# Autodesk Inventor assembly: CH_00_0000_gripper
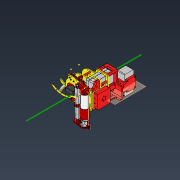
[picture p0: Inventor's stored thumbnail of the model, 180x180]
Saved by Autodesk Inventor 2022.3 (Build 263350030, 350C)
## iProperties
Created: 2022-02-10
Part Number: CH_00_0000_gripper
Document SubType Name: Assembly
Designer: Tomasz Krakowski
Author: Tomasz Krakowski
## Documents named in this file (57)
- C:\Repozytoria\sd-roboczy\01_praca\04_model\02_wykonawczy\CH_00_0000_gripper.iam
- C:\Repozytoria\sd-roboczy\01_praca\04_model\02_wykonawczy\CH_01_0001_base.ipt
- C:\Repozytoria\sd-roboczy\01_praca\04_model\02_wykonawczy\CH_01_0002_arm.ipt
- C:\Repozytoria\sd-roboczy\01_praca\04_model\02_wykonawczy\CH_01_0004_servo.ipt
- C:\Repozytoria\sd-roboczy\01_praca\04_model\02_wykonawczy\CH_01_0008_servo_horn.ipt
- C:\Repozytoria\sd-roboczy\01_praca\04_model\02_wykonawczy\CH_01_0006_syringe.ipt
- C:\Repozytoria\sd-roboczy\01_praca\04_model\02_wykonawczy\CH_01_0009_servo_shaft.ipt
- C:\Repozytoria\sd-roboczy\01_praca\04_model\02_wykonawczy\CH_01_0007_piston.ipt
- C:\Repozytoria\sd-roboczy\01_praca\04_model\02_wykonawczy\CH_01_0000_stem.ipt
- C:\Repozytoria\sd-roboczy\01_praca\04_model\02_wykonawczy\CH_01_0015_SKF_608_2RS1.ipt
- C:\Repozytoria\sd-roboczy\01_praca\04_model\02_wykonawczy\CH_01_0010_syringe_pump_servo.ipt
- C:\Repozytoria\sd-roboczy\01_praca\04_model\02_wykonawczy\CH_01_0012_bearing_plate.ipt
- C:\Repozytoria\sd-roboczy\01_praca\04_model\02_wykonawczy\CH_01_0014_syringe_mount_2.ipt
- C:\Repozytoria\sd-roboczy\01_praca\04_model\02_wykonawczy\CH_01_0016_syringe_mount_3.ipt
- C:\Repozytoria\sd-roboczy\01_praca\04_model\02_wykonawczy\CH_01_0017_distance.ipt
- C:\Repozytoria\sd-roboczy\01_praca\04_model\02_wykonawczy\CH_01_0018_arm.ipt
- C:\Repozytoria\sd-roboczy\01_praca\04_model\02_wykonawczy\CH_01_0019_bearing_plate_2.ipt
- C:\Repozytoria\sd-roboczy\01_praca\04_model\02_wykonawczy\CH_01_0020_servo_shaft_1.ipt
- C:\Repozytoria\sd-roboczy\01_praca\04_model\02_wykonawczy\CH_01_0021_distans_40mm.ipt
- C:\Repozytoria\sd-roboczy\01_praca\04_model\02_wykonawczy\CH_01_0025_end_switch.ipt
- C:\Repozytoria\sd-roboczy\01_praca\04_model\02_wykonawczy\CH_01_0025_end_switch_mount.ipt
- C:\Repozytoria\sd-roboczy\01_praca\04_model\02_wykonawczy\CH_01_0027_linear_actuator.ipt
- C:\Repozytoria\sd-roboczy\01_praca\04_model\02_wykonawczy\CH_01_0028_end_switch_mount_2.ipt
- C:\Repozytoria\sd-roboczy\01_praca\04_model\02_wykonawczy\CH_01_0029_syringe_pump_1.ipt
- C:\Repozytoria\sd-roboczy\01_praca\04_model\02_wykonawczy\CH_01_0022_bearing_mount.ipt
- C:\Repozytoria\sd-roboczy\01_praca\04_model\02_wykonawczy\CH_01_0031_bearing_mount_02.ipt
- C:\Repozytoria\sd-roboczy\01_praca\04_model\Content Center Files\en-US\DIN 912\DIN 912 - M3 x 0,5 x 8 x 6,75.ipt
- C:\Repozytoria\sd-roboczy\01_praca\04_model\Content Center Files\en-US\DIN 912\DIN 912 - M3 x 0,5 x 6 x 4,75.ipt
- C:\Repozytoria\sd-roboczy\01_praca\04_model\Content Center Files\en-US\DIN 912\DIN 912 - M3 x 0,5 x 16 x 14,75.ipt
- C:\Repozytoria\sd-roboczy\01_praca\04_model\Content Center Files\en-US\DIN 912\DIN 912 - M3 x 0,5 x 12 x 10,75.ipt
- C:\Repozytoria\sd-roboczy\01_praca\04_model\Content Center Files\en-US\PEM Concealed-head Standoffs CSS - Metric\CSS-M3-4.ipt
- C:\Repozytoria\sd-roboczy\01_praca\04_model\02_wykonawczy\CH_00_0001_needle_gripper.iam
- C:\Repozytoria\sd-roboczy\01_praca\04_model\02_wykonawczy\CH_01_0033_syringe_pump_nut_mount.ipt
- C:\Repozytoria\sd-roboczy\01_praca\04_model\02_wykonawczy\CH_01_0034_syringe_pump_nut_mount_2.ipt
- C:\Repozytoria\sd-roboczy\01_praca\04_model\Content Center Files\en-US\DIN 912\DIN 912 - M3 x 0.5 x 10 x 8.75.ipt
- C:\Repozytoria\sd-roboczy\01_praca\04_model\Content Center Files\en-US\DIN 912\DIN 912 - M3 x 0.5 x 6 x 4.75.ipt
- C:\Repozytoria\sd-roboczy\01_praca\04_model\02_wykonawczy\CH_01_0035_servo_mount.ipt
- C:\Repozytoria\sd-roboczy\01_praca\04_model\Content Center Files\en-US\DIN 912\DIN 912 - M4 x 0.7 x 8 x 6.25.ipt
- C:\Repozytoria\sd-roboczy\01_praca\04_model\Content Center Files\en-US\PEM Concealed-head Standoffs CSS - Metric\CSS-M4-4.ipt
- C:\Repozytoria\sd-roboczy\01_praca\04_model\Content Center Files\en-US\CNS 4433\CNS 4433 - M 2.ipt
- C:\Repozytoria\sd-roboczy\01_praca\04_model\Content Center Files\en-US\DIN 912\DIN 912 - M2 x 0.4 x 10 x 9.ipt
- C:\Repozytoria\sd-roboczy\01_praca\04_model\Content Center Files\en-US\DIN 912\DIN 912 - M4 x 0.7 x 40 x 20.ipt
- C:\Repozytoria\sd-roboczy\01_praca\04_model\02_wykonawczy\CH_00_0004_Z128.iam
- C:\Repozytoria\sd-roboczy\01_praca\04_model\02_wykonawczy\CH_01_0039_kradex_mount_1.ipt
- C:\Repozytoria\sd-roboczy\01_praca\04_model\02_wykonawczy\CH_01_0040_kradex_mount_2.ipt
- C:\Repozytoria\sd-roboczy\01_praca\04_model\02_wykonawczy\CH_01_0042_pcb_layout.ipt
- C:\Repozytoria\sd-roboczy\01_praca\04_model\02_wykonawczy\CH_01_0044_motor_end.ipt
- C:\Repozytoria\sd-roboczy\01_praca\04_model\02_wykonawczy\CH_01_0045_endefector_mount.ipt
- C:\Repozytoria\sd-roboczy\01_praca\04_model\02_wykonawczy\CH_01_0046_arm.ipt
- C:\Repozytoria\sd-roboczy\01_praca\04_model\02_wykonawczy\CH_01_0047_camera_mount.ipt
- C:\Repozytoria\sd-roboczy\01_praca\04_model\02_wykonawczy\CH_01_0043_camera_PH.ipt
- C:\Repozytoria\sd-roboczy\01_praca\04_model\02_wykonawczy\CH_01_0049_distans_40mm.ipt
- C:\Repozytoria\sd-roboczy\01_praca\04_model\02_wykonawczy\CH_01_0050_distans_40mm.ipt
- C:\Repozytoria\sd-roboczy\01_praca\04_model\02_wykonawczy\CH_01_0011_syringe_pump_needle mount_lower.ipt
- C:\Repozytoria\sd-roboczy\01_praca\04_model\02_wykonawczy\CH_01_0052_bracket_mount.ipt
- C:\Repozytoria\sd-roboczy\01_praca\04_model\02_wykonawczy\CH_01_0053_camera_mount.ipt
- C:\Repozytoria\sd-roboczy\01_praca\04_model\02_wykonawczy\CH_01_0054_camer_mount_part_b.ipt
## Components (121 placed, 55 different names)
1. CH_01_0001_base:1 — Mate:25, Mate:26, Mate:27, Zestawiający:43, pompa:51, Mate:53, Mate:54, Mate:58, Zestawiający:66, Zestawiający:73, Mate:94, Mate:100, Mate:102, Mate:103, Mate:106, Mate:115, Mate:164, Mate:165, Mate:166, Mate:169, Mate:170, Mate:171, Mate:172, Mate:179, Mate:180, Mate:181, Mate:182, Mate:193, Mate:194, Mate:196, Mate:225, Mate:226, Mate:289, Mate:290, Mate:292, Mate:295
2. CH_01_0002_arm:1 — Mate:17, Mate:18, Mate:19, Mate:30, Mate:32
3. CH_01_0006_syringe:1 — Mate:22, Mate:23, Zestawiający:49, Zestawiający:50, Mate:134, Mate:136
4. CH_01_0007_piston:1 — Mate:22, Mate:23, Mate:126, Mate:127, Mate:137, Flush:18
5. CH_01_0000_stem:1 — Mate:25
6. CH_01_0004_servo:1 — Mate:26, Mate:27, Mate:28, Mate:29, Mate:58
7. CH_01_0008_servo_horn:2 — Mate:28, Mate:29, Mate:30, Mate:31, Mate:32
8. SKF 2RS1-  with two seals SKF 2RS1608-2RS1:1 — Zestawiający:34, Mate:57, Mate:131
9. CH_01_0012_bearing_plate:1 — Zestawiający:43, Zestawiający:63, Zestawiający:64, Zestawiający:65, Zestawiający:66, Zestawiający:79, Zestawiający:80, Mate:101, Mate:110, Mate:112, Mate:113, Mate:114, Mate:132, Mate:133, Mate:233, Mate:234, Mate:235, Mate:236, Mate:237, Mate:238, Mate:246, Mate:251, Mate:252, Mate:253, Mate:254, Mate:259, Flush:48, Flush:49, Mate:281, Mate:282, Mate:283, Mate:284, Mate:285, Mate:286, Mate:287, Mate:288
10. CH_01_0014_syringe_mount_2:1 — Zestawiający:49, Zestawiający:50, pompa:51, Zestawiający:73, Mate:124, Mate:125, Mate:155, Flush:24, Mate:156, Flush:25, Mate:157
11. CH_01_0016_syringe_mount_3:1 — Mate:53, Mate:54, Mate:134, Mate:135, Flush:18, Mate:149, Mate:150, Mate:154, Flush:23, Mate:158, Mate:159
12. CH_01_0017_distance:1 — Mate:56, Mate:57, Zestawiający:62
13. CH_01_0018_arm:1 — Zestawiający:59, Zestawiający:60, Zestawiający:61
14. SKF 2RS1-  with two seals SKF 2RS1608-2RS1:2 — Zestawiający:62, Zestawiający:63, Równoległy:4, Mate:128, Mate:129
15. CH_01_0019_bearing_plate_2:1 — Zestawiający:64, Zestawiający:65, Równoległy:4, Zestawiający:82, Zestawiający:83, Mate:119, Mate:122, Flush:17, Mate:123, Mate:130, Mate:228, Mate:229, Mate:230, Mate:231, Mate:232, Mate:250, Mate:261, Mate:264, Mate:265, Mate:266, Mate:303, Flush:53, Flush:54
16. CH_01_0020_servo_shaft_1:1 — Zestawiający:67, Zestawiający:68, Mate:142
17. CH_01_0021_distans_40mm:3 — Zestawiający:79, Zestawiający:82, Mate:111, Flush:13
18. CH_01_0021_distans_40mm:4 — Zestawiający:80, Zestawiający:83, Mate:111, Flush:14
19. CH_01_0025_end_switch:1 — Mate:95, Mate:96, Mate:97, Mate:215, Mate:216, Mate:217
20. CH_01_0025_end_switch_mount:1 — Mate:94, Mate:95, Mate:96, Mate:97, Mate:102, Mate:103, Mate:177, Flush:28, Mate:178, Flush:29, Mate:202, Flush:35, Mate:203, Flush:36
21. CH_01_0027_linear_actuator:1 — Mate:124, Mate:125, Flush:25, Mate:296
22. CH_01_0021_distans_40mm:6 — Mate:100, Mate:101
23. CH_01_0028_end_switch_mount_2:1 — Mate:106, Mate:107, Mate:108, Mate:109, Mate:173, Flush:26, Mate:174, Flush:27, Mate:204, Mate:205, Flush:37, Flush:38
24. CH_01_0025_end_switch:2 — Mate:107, Mate:108, Mate:109, Mate:218, Mate:219, Mate:220
25. CH_01_0021_distans_40mm:7 — Mate:110, Flush:13, Mate:112, Mate:115
26. CH_01_0021_distans_40mm:8 — Mate:113, Flush:14, Mate:114
27. CH_01_0021_distans_40mm:9 — Mate:119, Mate:122, Mate:227
28. CH_01_0010_syringe_pump_servo:1 — Flush:17, Mate:123, Mate:246, Mate:267, Mate:268, Mate:269, Mate:298, Mate:299, Mate:300, Mate:301, Mate:302
29. CH_01_0029_syringe_pump_1:1 — Mate:126, Mate:127, Mate:137, Mate:143, Mate:145, Flush:20, Mate:297
30. CH_01_0022_bearing_mount:1 — Mate:128, Mate:129, Mate:130, Mate:221, Flush:41, Mate:222, Flush:42
31. CH_01_0031_bearing_mount_02:1 — Mate:131, Mate:132, Mate:133, Mate:223, Mate:224, Flush:43, Flush:44
32. DIN 912 - replaced by DIN EN ISO 4762 M3 x 8:1 — Mate:135, Mate:136
33. DIN 912 - replaced by DIN EN ISO 4762 M3 x 6:1 — Mate:143, Mate:152
34. DIN 912 - replaced by DIN EN ISO 4762 M3 x 6:2 — Mate:145, Mate:153
35. DIN 912 - replaced by DIN EN ISO 4762 M3 x 16:1 — Mate:296, Mate:297
36. DIN 912 - replaced by DIN EN ISO 4762 M3 x 12:1 — Mate:149, Mate:150, Mate:168
37. PEM Concealed-head Standoffs CSS - Metric CSS-M3-4:1 — Flush:20
38. PEM Concealed-head Standoffs CSS - Metric CSS-M3-4:3 — Mate:152
39. PEM Concealed-head Standoffs CSS - Metric CSS-M3-4:4 — Mate:153
40. PEM Concealed-head Standoffs CSS - Metric CSS-M3-4:5 — Mate:154, Flush:23
41. PEM Concealed-head Standoffs CSS - Metric CSS-M3-4:6 — Mate:155, Flush:24
42. DIN 912 - replaced by DIN EN ISO 4762 M3 x 16:3 — Mate:156, Mate:157
43. DIN 912 - replaced by DIN EN ISO 4762 M3 x 12:2 — Mate:158, Mate:159, Mate:167
44. DIN 912 - replaced by DIN EN ISO 4762 M3 x 10:2 — Mate:176
45. DIN 912 - replaced by DIN EN ISO 4762 M3 x 10:1 — Mate:175
46. CH_00_0001_needle_gripper:1 [sub-assembly] — Mate:164, Mate:165, Mate:166, Mate:185, Mate:186, Mate:187, Mate:188
47. CH_01_0033_syringe_pump_nut_mount:1 — Mate:167, Mate:168, Mate:169
48. CH_01_0034_syringe_pump_nut_mount_2:1 — Mate:170, Mate:171, Mate:172, Mate:183, Flush:30, Mate:184, Flush:31
49. PEM Concealed-head Standoffs CSS - Metric CSS-M3-4:7 — Mate:174, Flush:27, Mate:175
50. PEM Concealed-head Standoffs CSS - Metric CSS-M3-4:8 — Mate:173, Flush:26, Mate:176
51. PEM Concealed-head Standoffs CSS - Metric CSS-M3-4:9 — Mate:178, Flush:29
52. PEM Concealed-head Standoffs CSS - Metric CSS-M3-4:10 — Mate:177, Flush:28
53. DIN 912 - replaced by DIN EN ISO 4762 M3 x 6:3 — Mate:179, Mate:181
54. DIN 912 - replaced by DIN EN ISO 4762 M3 x 6:4 — Mate:180, Mate:182
55. PEM Concealed-head Standoffs CSS - Metric CSS-M3-4:11 — Mate:183, Flush:30
56. PEM Concealed-head Standoffs CSS - Metric CSS-M3-4:12 — Mate:184, Flush:31
57. DIN 912 - replaced by DIN EN ISO 4762 M3 x 10:3 — Mate:185, Mate:186, Mate:293
58. DIN 912 - replaced by DIN EN ISO 4762 M3 x 10:4 — Mate:187, Mate:188, Mate:294
59. CH_01_0035_servo_mount:1 — Mate:193, Mate:194, Mate:195, Mate:196, Flush:34
60. CNS 4433 M 2:1 — Mate:202, Flush:35
61. CNS 4433 M 2:3 — Mate:203, Flush:36
62. CNS 4433 M 2:4 — Mate:204, Flush:37
63. CNS 4433 M 2:5 — Mate:205, Flush:38
64. DIN 912 - replaced by DIN EN ISO 4762 M2 x 10:1 — Mate:215, Flush:39, Mate:217
65. DIN 912 - replaced by DIN EN ISO 4762 M2 x 10:2 — Mate:216, Flush:39
66. DIN 912 - replaced by DIN EN ISO 4762 M2 x 10:3 — Mate:218, Flush:40, Mate:220
67. DIN 912 - replaced by DIN EN ISO 4762 M2 x 10:4 — Mate:219, Flush:40
68. PEM Concealed-head Standoffs CSS - Metric CSS-M3-4:15 — Mate:221, Flush:41
69. PEM Concealed-head Standoffs CSS - Metric CSS-M3-4:16 — Mate:222, Flush:42
70. PEM Concealed-head Standoffs CSS - Metric CSS-M3-4:17 — Mate:223, Flush:43
71. PEM Concealed-head Standoffs CSS - Metric CSS-M3-4:18 — Mate:224, Flush:44
72. DIN 912 - replaced by DIN EN ISO 4762 M3 x 6:9 — Mate:225, Mate:226
73. DIN 912 - replaced by DIN EN ISO 4762 M3 x 6:14 — Mate:229, Mate:230
74. DIN 912 - replaced by DIN EN ISO 4762 M3 x 6:15 — Mate:231, Mate:232
75. DIN 912 - replaced by DIN EN ISO 4762 M3 x 6:16 — Mate:233, Flush:45
76. DIN 912 - replaced by DIN EN ISO 4762 M3 x 6:17 — Mate:234, Flush:45, Mate:235
77. CH_00_0001_needle_gripper:2 [sub-assembly] — Mate:236, Mate:237, Mate:238
78. CH_00_0004_Z128:1 [sub-assembly] — Mate:261, Mate:262, Flush:50, Mate:263, Mate:266, Flush:51
79. CH_01_0039_kradex_mount_1:1 — Mate:250, Mate:255, Mate:256, Mate:257, Flush:51
80. DIN 912 - replaced by DIN EN ISO 4762 M3 x 10:5 — Mate:251, Mate:253
81. DIN 912 - replaced by DIN EN ISO 4762 M3 x 10:6 — Mate:252, Mate:254
82. DIN 912 - replaced by DIN EN ISO 4762 M3 x 10:7 — Mate:255, Flush:47, Mate:264
83. DIN 912 - replaced by DIN EN ISO 4762 M3 x 10:8 — Mate:256, Flush:47, Mate:257, Mate:265
84. CH_01_0040_kradex_mount_2:1 — Mate:259, Flush:48, Flush:49
85. CH_01_0042_pcb_layout:1 — Mate:262, Flush:50, Mate:263
86. CH_01_0044_motor_end:1 — Mate:270, Mate:271, Mate:272, Mate:273, Mate:274, Mate:277, Mate:278
87. CH_01_0045_endefector_mount:1 — Mate:267, Mate:268, Mate:269, Mate:270, Mate:271, Mate:272
88. CH_01_0046_arm:1 — Mate:273, Mate:274, Mate:275, Mate:276, Mate:277
89. CH_01_0047_camera_mount:1 — Mate:275, Mate:276, Mate:278
90. CH_01_0043_camera_PH:1 — Mate:304, Mate:305, Mate:306
91. CH_01_0049_distans_40mm:1 — Mate:281, Mate:287
92. CH_01_0049_distans_40mm:2 — Mate:282, Mate:288
93. CH_01_0049_distans_40mm:3 — Mate:283, Mate:284
94. CH_01_0049_distans_40mm:4 — Mate:285, Mate:286
95. CH_01_0050_distans_40mm:1 — Mate:290, Mate:291, Mate:292
96. CH_01_0050_distans_40mm:2 — Mate:289, Mate:291
97. CH_01_0011_syringe_pump_needle mount_lower:1 — Mate:293, Mate:294, Mate:295
98. CH_01_0052_bracket_mount:1 — Mate:298, Mate:301
99. CH_01_0052_bracket_mount:2 — Mate:299, Mate:300, Mate:302
100. CH_01_0053_camera_mount:1 — Mate:303, Flush:53, Flush:54, Mate:307, Mate:308
101. CH_01_0054_camer_mount_part_b:1 — Mate:304, Mate:305, Mate:306, Mate:307, Mate:308
102. DIN 912 - replaced by DIN EN ISO 4762 M3 x 6:5 — Mate:191, Mate:192
103. CH_01_0009_servo_shaft:1 — Mate:17, Mate:18, Mate:19, Mate:31, Zestawiający:34, Mate:56, Zestawiający:59, Zestawiający:60, Zestawiający:61, Zestawiający:67, Zestawiający:68, Mate:142, Mate:191, Mate:192
104. DIN 912 - replaced by DIN EN ISO 4762 M3 x 6:6
105. CH_01_0009_servo_shaft:2
106. DIN 912 - replaced by DIN EN ISO 4762 M3 x 6:7
107. CH_01_0009_servo_shaft:3
108. DIN 912 - replaced by DIN EN ISO 4762 M3 x 6:8
109. CH_01_0009_servo_shaft:4
110. PEM Concealed-head Standoffs CSS - Metric CSS-M4-4:1 — Mate:195, Flush:34
111. PEM Concealed-head Standoffs CSS - Metric CSS-M4-4:2
112. PEM Concealed-head Standoffs CSS - Metric CSS-M4-4:3
113. PEM Concealed-head Standoffs CSS - Metric CSS-M4-4:4
114. DIN 912 - replaced by DIN EN ISO 4762 M4 x 8:1
115. DIN 912 - replaced by DIN EN ISO 4762 M4 x 8:2
116. DIN 912 - replaced by DIN EN ISO 4762 M4 x 8:3
117. DIN 912 - replaced by DIN EN ISO 4762 M4 x 8:4
118. DIN 912 - replaced by DIN EN ISO 4762 M4 x 40:1 — Mate:227, Mate:228
119. DIN 912 - replaced by DIN EN ISO 4762 M4 x 40:2
120. DIN 912 - replaced by DIN EN ISO 4762 M4 x 40:3
121. DIN 912 - replaced by DIN EN ISO 4762 M4 x 40:4
## Component patterns: (4 elements, first: DIN 912 - replaced by DIN EN ISO 4762 M3 x 6:5 + CH_01_0009_servo_shaft:1), (4 elements, first: PEM Concealed-head Standoffs CSS - Metric CSS-M4-4:1), (4 elements, first: DIN 912 - replaced by DIN EN ISO 4762 M4 x 8:1), (4 elements, first: DIN 912 - replaced by DIN EN ISO 4762 M4 x 40:1)
## Relationships (240: Mate 206, Flush 34)
- Mate:17: CH_01_0002_arm:1 ↔ CH_01_0009_servo_shaft:1
- Mate:18: CH_01_0002_arm:1 ↔ CH_01_0009_servo_shaft:1
- Mate:19: CH_01_0002_arm:1 ↔ CH_01_0009_servo_shaft:1
- Mate:22: CH_01_0006_syringe:1 ↔ CH_01_0007_piston:1
- Mate:23: CH_01_0006_syringe:1 ↔ CH_01_0007_piston:1
- Mate:25: CH_01_0001_base:1 ↔ CH_01_0000_stem:1
- Mate:26: CH_01_0001_base:1 ↔ CH_01_0004_servo:1
- Mate:27: CH_01_0001_base:1 ↔ CH_01_0004_servo:1
- Mate:28: CH_01_0004_servo:1 ↔ CH_01_0008_servo_horn:2
- Mate:29: CH_01_0004_servo:1 ↔ CH_01_0008_servo_horn:2
- Mate:30: CH_01_0002_arm:1 ↔ CH_01_0008_servo_horn:2
- Mate:31: CH_01_0008_servo_horn:2 ↔ CH_01_0009_servo_shaft:1
- Mate:32: CH_01_0002_arm:1 ↔ CH_01_0008_servo_horn:2
- Zestawiający:34 [Mate]: SKF 2RS1-  with two seals SKF 2RS1608-2RS1:1 ↔ CH_01_0009_servo_shaft:1
- Zestawiający:43 [Mate]: CH_01_0001_base:1 ↔ CH_01_0012_bearing_plate:1
- Zestawiający:49 [Mate]: CH_01_0006_syringe:1 ↔ CH_01_0014_syringe_mount_2:1
- Zestawiający:50 [Mate]: CH_01_0006_syringe:1 ↔ CH_01_0014_syringe_mount_2:1
- pompa:51 [Mate] (4 mm): CH_01_0001_base:1 ↔ CH_01_0014_syringe_mount_2:1
- Mate:53: CH_01_0001_base:1 ↔ CH_01_0016_syringe_mount_3:1
- Mate:54: CH_01_0001_base:1 ↔ CH_01_0016_syringe_mount_3:1
- Mate:56: CH_01_0017_distance:1 ↔ CH_01_0009_servo_shaft:1
- Mate:57: SKF 2RS1-  with two seals SKF 2RS1608-2RS1:1 ↔ CH_01_0017_distance:1
- Mate:58: CH_01_0001_base:1 ↔ CH_01_0004_servo:1
- Zestawiający:59 [Mate]: CH_01_0018_arm:1 ↔ CH_01_0009_servo_shaft:1
- Zestawiający:60 [Mate]: CH_01_0018_arm:1 ↔ CH_01_0009_servo_shaft:1
- Zestawiający:61 [Mate]: CH_01_0018_arm:1 ↔ CH_01_0009_servo_shaft:1
- Zestawiający:62 [Mate]: CH_01_0017_distance:1 ↔ SKF 2RS1-  with two seals SKF 2RS1608-2RS1:2
- Zestawiający:63 [Mate] (40 mm): CH_01_0012_bearing_plate:1 ↔ SKF 2RS1-  with two seals SKF 2RS1608-2RS1:2
- Zestawiający:64 [Mate]: CH_01_0012_bearing_plate:1 ↔ CH_01_0019_bearing_plate_2:1
- Zestawiający:65 [Mate]: CH_01_0012_bearing_plate:1 ↔ CH_01_0019_bearing_plate_2:1
- Zestawiający:66 [Mate]: CH_01_0001_base:1 ↔ CH_01_0012_bearing_plate:1
- Równoległy:4 [Flush]: SKF 2RS1-  with two seals SKF 2RS1608-2RS1:2 ↔ CH_01_0019_bearing_plate_2:1
- Zestawiający:67 [Mate]: CH_01_0020_servo_shaft_1:1 ↔ CH_01_0009_servo_shaft:1
- Zestawiający:68 [Mate]: CH_01_0020_servo_shaft_1:1 ↔ CH_01_0009_servo_shaft:1
- Zestawiający:73 [Mate]: CH_01_0001_base:1 ↔ CH_01_0014_syringe_mount_2:1
- Zestawiający:79 [Mate]: CH_01_0012_bearing_plate:1 ↔ CH_01_0021_distans_40mm:3
- Zestawiający:80 [Mate]: CH_01_0012_bearing_plate:1 ↔ CH_01_0021_distans_40mm:4
- Zestawiający:82 [Mate]: CH_01_0019_bearing_plate_2:1 ↔ CH_01_0021_distans_40mm:3
- Zestawiający:83 [Mate]: CH_01_0019_bearing_plate_2:1 ↔ CH_01_0021_distans_40mm:4
- Mate:94: CH_01_0001_base:1 ↔ CH_01_0025_end_switch_mount:1
- Mate:95: CH_01_0025_end_switch:1 ↔ CH_01_0025_end_switch_mount:1
- Mate:96: CH_01_0025_end_switch:1 ↔ CH_01_0025_end_switch_mount:1
- Mate:97: CH_01_0025_end_switch:1 ↔ CH_01_0025_end_switch_mount:1
- Mate:100: CH_01_0001_base:1 ↔ CH_01_0021_distans_40mm:6
- Mate:101: CH_01_0012_bearing_plate:1 ↔ CH_01_0021_distans_40mm:6
- Mate:102: CH_01_0001_base:1 ↔ CH_01_0025_end_switch_mount:1
- Mate:103: CH_01_0001_base:1 ↔ CH_01_0025_end_switch_mount:1
- Mate:106: CH_01_0001_base:1 ↔ CH_01_0028_end_switch_mount_2:1
- Mate:107: CH_01_0028_end_switch_mount_2:1 ↔ CH_01_0025_end_switch:2
- Mate:108: CH_01_0028_end_switch_mount_2:1 ↔ CH_01_0025_end_switch:2
- Mate:109: CH_01_0028_end_switch_mount_2:1 ↔ CH_01_0025_end_switch:2
- Mate:110: CH_01_0012_bearing_plate:1 ↔ CH_01_0021_distans_40mm:7
- Mate:111: CH_01_0021_distans_40mm:3 ↔ CH_01_0021_distans_40mm:4
- Flush:13: CH_01_0021_distans_40mm:3 ↔ CH_01_0021_distans_40mm:7
- Mate:112: CH_01_0012_bearing_plate:1 ↔ CH_01_0021_distans_40mm:7
- Mate:113: CH_01_0012_bearing_plate:1 ↔ CH_01_0021_distans_40mm:8
- Flush:14: CH_01_0021_distans_40mm:4 ↔ CH_01_0021_distans_40mm:8
- Mate:114: CH_01_0012_bearing_plate:1 ↔ CH_01_0021_distans_40mm:8
- Mate:115: CH_01_0001_base:1 ↔ CH_01_0021_distans_40mm:7
- Mate:119: CH_01_0019_bearing_plate_2:1 ↔ CH_01_0021_distans_40mm:9
- Mate:122: CH_01_0019_bearing_plate_2:1 ↔ CH_01_0021_distans_40mm:9
- Flush:17: CH_01_0019_bearing_plate_2:1 ↔ CH_01_0010_syringe_pump_servo:1
- Mate:123: CH_01_0019_bearing_plate_2:1 ↔ CH_01_0010_syringe_pump_servo:1
- Mate:124: CH_01_0014_syringe_mount_2:1 ↔ CH_01_0027_linear_actuator:1
- Mate:125: CH_01_0014_syringe_mount_2:1 ↔ CH_01_0027_linear_actuator:1
- Mate:126: CH_01_0007_piston:1 ↔ CH_01_0029_syringe_pump_1:1
- Mate:127: CH_01_0007_piston:1 ↔ CH_01_0029_syringe_pump_1:1
- Mate:128: SKF 2RS1-  with two seals SKF 2RS1608-2RS1:2 ↔ CH_01_0022_bearing_mount:1
- Mate:129: SKF 2RS1-  with two seals SKF 2RS1608-2RS1:2 ↔ CH_01_0022_bearing_mount:1
- Mate:130: CH_01_0019_bearing_plate_2:1 ↔ CH_01_0022_bearing_mount:1
- Mate:131: SKF 2RS1-  with two seals SKF 2RS1608-2RS1:1 ↔ CH_01_0031_bearing_mount_02:1
- Mate:132: CH_01_0012_bearing_plate:1 ↔ CH_01_0031_bearing_mount_02:1
- Mate:133: CH_01_0012_bearing_plate:1 ↔ CH_01_0031_bearing_mount_02:1
- Mate:134: CH_01_0006_syringe:1 ↔ CH_01_0016_syringe_mount_3:1
- Mate:135: CH_01_0016_syringe_mount_3:1 ↔ DIN 912 - replaced by DIN EN ISO 4762 M3 x 8:1
- Mate:136: CH_01_0006_syringe:1 ↔ DIN 912 - replaced by DIN EN ISO 4762 M3 x 8:1
- Mate:137: CH_01_0007_piston:1 ↔ CH_01_0029_syringe_pump_1:1
- Flush:18: CH_01_0007_piston:1 ↔ CH_01_0016_syringe_mount_3:1
- Mate:142: CH_01_0020_servo_shaft_1:1 ↔ CH_01_0009_servo_shaft:1
- Mate:143: CH_01_0029_syringe_pump_1:1 ↔ DIN 912 - replaced by DIN EN ISO 4762 M3 x 6:1
- Mate:145: CH_01_0029_syringe_pump_1:1 ↔ DIN 912 - replaced by DIN EN ISO 4762 M3 x 6:2
- Mate:149: CH_01_0016_syringe_mount_3:1 ↔ DIN 912 - replaced by DIN EN ISO 4762 M3 x 12:1
- Mate:150: CH_01_0016_syringe_mount_3:1 ↔ DIN 912 - replaced by DIN EN ISO 4762 M3 x 12:1
- Flush:20 (0.1 mm): CH_01_0029_syringe_pump_1:1 ↔ PEM Concealed-head Standoffs CSS - Metric CSS-M3-4:1
- Mate:152: DIN 912 - replaced by DIN EN ISO 4762 M3 x 6:1 ↔ PEM Concealed-head Standoffs CSS - Metric CSS-M3-4:3
- Mate:153: DIN 912 - replaced by DIN EN ISO 4762 M3 x 6:2 ↔ PEM Concealed-head Standoffs CSS - Metric CSS-M3-4:4
- Mate:154: CH_01_0016_syringe_mount_3:1 ↔ PEM Concealed-head Standoffs CSS - Metric CSS-M3-4:5
- Flush:23 (0.1 mm): CH_01_0016_syringe_mount_3:1 ↔ PEM Concealed-head Standoffs CSS - Metric CSS-M3-4:5
- Mate:155: CH_01_0014_syringe_mount_2:1 ↔ PEM Concealed-head Standoffs CSS - Metric CSS-M3-4:6
- Flush:24 (0.1 mm): CH_01_0014_syringe_mount_2:1 ↔ PEM Concealed-head Standoffs CSS - Metric CSS-M3-4:6
- Mate:156: CH_01_0014_syringe_mount_2:1 ↔ DIN 912 - replaced by DIN EN ISO 4762 M3 x 16:3
- Flush:25: CH_01_0014_syringe_mount_2:1 ↔ CH_01_0027_linear_actuator:1
- Mate:157: CH_01_0014_syringe_mount_2:1 ↔ DIN 912 - replaced by DIN EN ISO 4762 M3 x 16:3
- Mate:158: CH_01_0016_syringe_mount_3:1 ↔ DIN 912 - replaced by DIN EN ISO 4762 M3 x 12:2
- Mate:159: CH_01_0016_syringe_mount_3:1 ↔ DIN 912 - replaced by DIN EN ISO 4762 M3 x 12:2
- [Mate]: CH_01_0014_syringe_mount_2:1 ↔ DIN 912 - replaced by DIN EN ISO 4762 M3 x 10:1
- [Mate]: CH_01_0014_syringe_mount_2:1 ↔ DIN 912 - replaced by DIN EN ISO 4762 M3 x 10:2
- [Mate]: CH_01_0014_syringe_mount_2:1 ↔ DIN 912 - replaced by DIN EN ISO 4762 M3 x 10:1
- [Mate]: CH_01_0014_syringe_mount_2:1 ↔ DIN 912 - replaced by DIN EN ISO 4762 M3 x 10:2
- Mate:164: CH_01_0001_base:1 ↔ CH_00_0001_needle_gripper:1
- Mate:165: CH_01_0001_base:1 ↔ CH_00_0001_needle_gripper:1
- Mate:166: CH_01_0001_base:1 ↔ CH_00_0001_needle_gripper:1
- Mate:167: DIN 912 - replaced by DIN EN ISO 4762 M3 x 12:2 ↔ CH_01_0033_syringe_pump_nut_mount:1
- Mate:168: DIN 912 - replaced by DIN EN ISO 4762 M3 x 12:1 ↔ CH_01_0033_syringe_pump_nut_mount:1
- Mate:169: CH_01_0001_base:1 ↔ CH_01_0033_syringe_pump_nut_mount:1
- Mate:170: CH_01_0001_base:1 ↔ CH_01_0034_syringe_pump_nut_mount_2:1
- Mate:171: CH_01_0001_base:1 ↔ CH_01_0034_syringe_pump_nut_mount_2:1
- Mate:172: CH_01_0001_base:1 ↔ CH_01_0034_syringe_pump_nut_mount_2:1
- Mate:173: CH_01_0028_end_switch_mount_2:1 ↔ PEM Concealed-head Standoffs CSS - Metric CSS-M3-4:8
- Flush:26 (0.1 mm): CH_01_0028_end_switch_mount_2:1 ↔ PEM Concealed-head Standoffs CSS - Metric CSS-M3-4:8
- Mate:174: CH_01_0028_end_switch_mount_2:1 ↔ PEM Concealed-head Standoffs CSS - Metric CSS-M3-4:7
- Flush:27 (0.1 mm): CH_01_0028_end_switch_mount_2:1 ↔ PEM Concealed-head Standoffs CSS - Metric CSS-M3-4:7
- Mate:175: DIN 912 - replaced by DIN EN ISO 4762 M3 x 10:1 ↔ PEM Concealed-head Standoffs CSS - Metric CSS-M3-4:7
- Mate:176: DIN 912 - replaced by DIN EN ISO 4762 M3 x 10:2 ↔ PEM Concealed-head Standoffs CSS - Metric CSS-M3-4:8
- Mate:177: CH_01_0025_end_switch_mount:1 ↔ PEM Concealed-head Standoffs CSS - Metric CSS-M3-4:10
- Flush:28 (0.1 mm): CH_01_0025_end_switch_mount:1 ↔ PEM Concealed-head Standoffs CSS - Metric CSS-M3-4:10
- Mate:178: CH_01_0025_end_switch_mount:1 ↔ PEM Concealed-head Standoffs CSS - Metric CSS-M3-4:9
- Flush:29 (0.1 mm): CH_01_0025_end_switch_mount:1 ↔ PEM Concealed-head Standoffs CSS - Metric CSS-M3-4:9
- Mate:179: CH_01_0001_base:1 ↔ DIN 912 - replaced by DIN EN ISO 4762 M3 x 6:3
- Mate:180: CH_01_0001_base:1 ↔ DIN 912 - replaced by DIN EN ISO 4762 M3 x 6:4
- Mate:181: CH_01_0001_base:1 ↔ DIN 912 - replaced by DIN EN ISO 4762 M3 x 6:3
- Mate:182: CH_01_0001_base:1 ↔ DIN 912 - replaced by DIN EN ISO 4762 M3 x 6:4
- Mate:183: CH_01_0034_syringe_pump_nut_mount_2:1 ↔ PEM Concealed-head Standoffs CSS - Metric CSS-M3-4:11
- Flush:30 (0.1 mm): CH_01_0034_syringe_pump_nut_mount_2:1 ↔ PEM Concealed-head Standoffs CSS - Metric CSS-M3-4:11
- Mate:184: CH_01_0034_syringe_pump_nut_mount_2:1 ↔ PEM Concealed-head Standoffs CSS - Metric CSS-M3-4:12
- Flush:31 (0.1 mm): CH_01_0034_syringe_pump_nut_mount_2:1 ↔ PEM Concealed-head Standoffs CSS - Metric CSS-M3-4:12
- Mate:185: CH_00_0001_needle_gripper:1 ↔ DIN 912 - replaced by DIN EN ISO 4762 M3 x 10:3
- Mate:186: CH_00_0001_needle_gripper:1 ↔ DIN 912 - replaced by DIN EN ISO 4762 M3 x 10:3
- Mate:187: CH_00_0001_needle_gripper:1 ↔ DIN 912 - replaced by DIN EN ISO 4762 M3 x 10:4
- Mate:188: CH_00_0001_needle_gripper:1 ↔ DIN 912 - replaced by DIN EN ISO 4762 M3 x 10:4
- Mate:191: DIN 912 - replaced by DIN EN ISO 4762 M3 x 6:5 ↔ CH_01_0009_servo_shaft:1
- Mate:192: DIN 912 - replaced by DIN EN ISO 4762 M3 x 6:5 ↔ CH_01_0009_servo_shaft:1
- Mate:193: CH_01_0001_base:1 ↔ CH_01_0035_servo_mount:1
- Mate:194: CH_01_0001_base:1 ↔ CH_01_0035_servo_mount:1
- Mate:195: CH_01_0035_servo_mount:1 ↔ PEM Concealed-head Standoffs CSS - Metric CSS-M4-4:1
- Mate:196: CH_01_0001_base:1 ↔ CH_01_0035_servo_mount:1
- Flush:34 (0.1 mm): CH_01_0035_servo_mount:1 ↔ PEM Concealed-head Standoffs CSS - Metric CSS-M4-4:1
- [Mate]: CH_01_0001_base:1 ↔ DIN 912 - replaced by DIN EN ISO 4762 M4 x 8:1
- Mate:202: CH_01_0025_end_switch_mount:1 ↔ CNS 4433 M 2:1
- Flush:35 (0.1 mm): CH_01_0025_end_switch_mount:1 ↔ CNS 4433 M 2:1
- Mate:203: CH_01_0025_end_switch_mount:1 ↔ CNS 4433 M 2:3
- Flush:36 (0.1 mm): CH_01_0025_end_switch_mount:1 ↔ CNS 4433 M 2:3
- Mate:204: CH_01_0028_end_switch_mount_2:1 ↔ CNS 4433 M 2:4
- Mate:205: CH_01_0028_end_switch_mount_2:1 ↔ CNS 4433 M 2:5
- Flush:37 (0.1 mm): CH_01_0028_end_switch_mount_2:1 ↔ CNS 4433 M 2:4
- Flush:38 (0.1 mm): CH_01_0028_end_switch_mount_2:1 ↔ CNS 4433 M 2:5
- Mate:215: CH_01_0025_end_switch:1 ↔ DIN 912 - replaced by DIN EN ISO 4762 M2 x 10:1
- Mate:216: CH_01_0025_end_switch:1 ↔ DIN 912 - replaced by DIN EN ISO 4762 M2 x 10:2
- Flush:39: DIN 912 - replaced by DIN EN ISO 4762 M2 x 10:1 ↔ DIN 912 - replaced by DIN EN ISO 4762 M2 x 10:2
- Mate:217: CH_01_0025_end_switch:1 ↔ DIN 912 - replaced by DIN EN ISO 4762 M2 x 10:1
- Mate:218: CH_01_0025_end_switch:2 ↔ DIN 912 - replaced by DIN EN ISO 4762 M2 x 10:3
- Mate:219: CH_01_0025_end_switch:2 ↔ DIN 912 - replaced by DIN EN ISO 4762 M2 x 10:4
- Flush:40: DIN 912 - replaced by DIN EN ISO 4762 M2 x 10:3 ↔ DIN 912 - replaced by DIN EN ISO 4762 M2 x 10:4
- Mate:220: CH_01_0025_end_switch:2 ↔ DIN 912 - replaced by DIN EN ISO 4762 M2 x 10:3
- Mate:221: CH_01_0022_bearing_mount:1 ↔ PEM Concealed-head Standoffs CSS - Metric CSS-M3-4:15
- Flush:41 (0.1 mm): CH_01_0022_bearing_mount:1 ↔ PEM Concealed-head Standoffs CSS - Metric CSS-M3-4:15
- Mate:222: CH_01_0022_bearing_mount:1 ↔ PEM Concealed-head Standoffs CSS - Metric CSS-M3-4:16
- Flush:42 (0.1 mm): CH_01_0022_bearing_mount:1 ↔ PEM Concealed-head Standoffs CSS - Metric CSS-M3-4:16
- Mate:223: CH_01_0031_bearing_mount_02:1 ↔ PEM Concealed-head Standoffs CSS - Metric CSS-M3-4:17
- Mate:224: CH_01_0031_bearing_mount_02:1 ↔ PEM Concealed-head Standoffs CSS - Metric CSS-M3-4:18
- Flush:43 (0.1 mm): CH_01_0031_bearing_mount_02:1 ↔ PEM Concealed-head Standoffs CSS - Metric CSS-M3-4:17
- Flush:44 (0.1 mm): CH_01_0031_bearing_mount_02:1 ↔ PEM Concealed-head Standoffs CSS - Metric CSS-M3-4:18
- Mate:225: CH_01_0001_base:1 ↔ DIN 912 - replaced by DIN EN ISO 4762 M3 x 6:9
- Mate:226: CH_01_0001_base:1 ↔ DIN 912 - replaced by DIN EN ISO 4762 M3 x 6:9
- Mate:227: CH_01_0021_distans_40mm:9 ↔ DIN 912 - replaced by DIN EN ISO 4762 M4 x 40:1
- Mate:228: CH_01_0019_bearing_plate_2:1 ↔ DIN 912 - replaced by DIN EN ISO 4762 M4 x 40:1
- Mate:229: CH_01_0019_bearing_plate_2:1 ↔ DIN 912 - replaced by DIN EN ISO 4762 M3 x 6:14
- Mate:230: CH_01_0019_bearing_plate_2:1 ↔ DIN 912 - replaced by DIN EN ISO 4762 M3 x 6:14
- Mate:231: CH_01_0019_bearing_plate_2:1 ↔ DIN 912 - replaced by DIN EN ISO 4762 M3 x 6:15
- Mate:232: CH_01_0019_bearing_plate_2:1 ↔ DIN 912 - replaced by DIN EN ISO 4762 M3 x 6:15
- Mate:233: CH_01_0012_bearing_plate:1 ↔ DIN 912 - replaced by DIN EN ISO 4762 M3 x 6:16
- Mate:234: CH_01_0012_bearing_plate:1 ↔ DIN 912 - replaced by DIN EN ISO 4762 M3 x 6:17
- Flush:45: DIN 912 - replaced by DIN EN ISO 4762 M3 x 6:16 ↔ DIN 912 - replaced by DIN EN ISO 4762 M3 x 6:17
- Mate:235: CH_01_0012_bearing_plate:1 ↔ DIN 912 - replaced by DIN EN ISO 4762 M3 x 6:17
- Mate:236: CH_01_0012_bearing_plate:1 ↔ CH_00_0001_needle_gripper:2
- Mate:237: CH_01_0012_bearing_plate:1 ↔ CH_00_0001_needle_gripper:2
- Mate:238: CH_01_0012_bearing_plate:1 ↔ CH_00_0001_needle_gripper:2
- Mate:246: CH_01_0012_bearing_plate:1 ↔ CH_01_0010_syringe_pump_servo:1
- Mate:250: CH_01_0019_bearing_plate_2:1 ↔ CH_01_0039_kradex_mount_1:1
- Mate:251: CH_01_0012_bearing_plate:1 ↔ DIN 912 - replaced by DIN EN ISO 4762 M3 x 10:5
- Mate:252: CH_01_0012_bearing_plate:1 ↔ DIN 912 - replaced by DIN EN ISO 4762 M3 x 10:6
- Mate:253: CH_01_0012_bearing_plate:1 ↔ DIN 912 - replaced by DIN EN ISO 4762 M3 x 10:5
- Mate:254: CH_01_0012_bearing_plate:1 ↔ DIN 912 - replaced by DIN EN ISO 4762 M3 x 10:6
- Mate:255: CH_01_0039_kradex_mount_1:1 ↔ DIN 912 - replaced by DIN EN ISO 4762 M3 x 10:7
- Mate:256: CH_01_0039_kradex_mount_1:1 ↔ DIN 912 - replaced by DIN EN ISO 4762 M3 x 10:8
- Flush:47: DIN 912 - replaced by DIN EN ISO 4762 M3 x 10:7 ↔ DIN 912 - replaced by DIN EN ISO 4762 M3 x 10:8
- Mate:257: CH_01_0039_kradex_mount_1:1 ↔ DIN 912 - replaced by DIN EN ISO 4762 M3 x 10:8
- Mate:259: CH_01_0012_bearing_plate:1 ↔ CH_01_0040_kradex_mount_2:1
- Flush:48: CH_01_0012_bearing_plate:1 ↔ CH_01_0040_kradex_mount_2:1
- Flush:49: CH_01_0012_bearing_plate:1 ↔ CH_01_0040_kradex_mount_2:1
- Mate:261 (37 mm): CH_01_0019_bearing_plate_2:1 ↔ CH_00_0004_Z128:1
- Mate:262: CH_00_0004_Z128:1 ↔ CH_01_0042_pcb_layout:1
- Flush:50: CH_00_0004_Z128:1 ↔ CH_01_0042_pcb_layout:1
- Mate:263: CH_00_0004_Z128:1 ↔ CH_01_0042_pcb_layout:1
- Mate:264: CH_01_0019_bearing_plate_2:1 ↔ DIN 912 - replaced by DIN EN ISO 4762 M3 x 10:7
- Mate:265: CH_01_0019_bearing_plate_2:1 ↔ DIN 912 - replaced by DIN EN ISO 4762 M3 x 10:8
- Mate:266: CH_01_0019_bearing_plate_2:1 ↔ CH_00_0004_Z128:1
- Flush:51 (52.7 mm): CH_00_0004_Z128:1 ↔ CH_01_0039_kradex_mount_1:1
- Mate:267: CH_01_0010_syringe_pump_servo:1 ↔ CH_01_0045_endefector_mount:1
- Mate:268: CH_01_0010_syringe_pump_servo:1 ↔ CH_01_0045_endefector_mount:1
- Mate:269: CH_01_0010_syringe_pump_servo:1 ↔ CH_01_0045_endefector_mount:1
- Mate:270: CH_01_0044_motor_end:1 ↔ CH_01_0045_endefector_mount:1
- Mate:271: CH_01_0044_motor_end:1 ↔ CH_01_0045_endefector_mount:1
- Mate:272: CH_01_0044_motor_end:1 ↔ CH_01_0045_endefector_mount:1
- Mate:273: CH_01_0044_motor_end:1 ↔ CH_01_0046_arm:1
- Mate:274: CH_01_0044_motor_end:1 ↔ CH_01_0046_arm:1
- Mate:275: CH_01_0046_arm:1 ↔ CH_01_0047_camera_mount:1
- Mate:276: CH_01_0046_arm:1 ↔ CH_01_0047_camera_mount:1
- Mate:277: CH_01_0044_motor_end:1 ↔ CH_01_0046_arm:1
- Mate:278 (250 mm): CH_01_0044_motor_end:1 ↔ CH_01_0047_camera_mount:1
- Mate:281: CH_01_0012_bearing_plate:1 ↔ CH_01_0049_distans_40mm:1
- Mate:282: CH_01_0012_bearing_plate:1 ↔ CH_01_0049_distans_40mm:2
- Mate:283: CH_01_0012_bearing_plate:1 ↔ CH_01_0049_distans_40mm:3
- Mate:284: CH_01_0012_bearing_plate:1 ↔ CH_01_0049_distans_40mm:3
- Mate:285: CH_01_0012_bearing_plate:1 ↔ CH_01_0049_distans_40mm:4
- Mate:286: CH_01_0012_bearing_plate:1 ↔ CH_01_0049_distans_40mm:4
- Mate:287: CH_01_0012_bearing_plate:1 ↔ CH_01_0049_distans_40mm:1
- Mate:288: CH_01_0012_bearing_plate:1 ↔ CH_01_0049_distans_40mm:2
- Mate:289: CH_01_0001_base:1 ↔ CH_01_0050_distans_40mm:2
- Mate:290: CH_01_0001_base:1 ↔ CH_01_0050_distans_40mm:1
- Mate:291: CH_01_0050_distans_40mm:1 ↔ CH_01_0050_distans_40mm:2
- Mate:292: CH_01_0001_base:1 ↔ CH_01_0050_distans_40mm:1
- Mate:293: DIN 912 - replaced by DIN EN ISO 4762 M3 x 10:3 ↔ CH_01_0011_syringe_pump_needle mount_lower:1
- Mate:294: DIN 912 - replaced by DIN EN ISO 4762 M3 x 10:4 ↔ CH_01_0011_syringe_pump_needle mount_lower:1
- Mate:295: CH_01_0001_base:1 ↔ CH_01_0011_syringe_pump_needle mount_lower:1
- Mate:296: CH_01_0027_linear_actuator:1 ↔ DIN 912 - replaced by DIN EN ISO 4762 M3 x 16:1
- Mate:297: CH_01_0029_syringe_pump_1:1 ↔ DIN 912 - replaced by DIN EN ISO 4762 M3 x 16:1
- Mate:298: CH_01_0010_syringe_pump_servo:1 ↔ CH_01_0052_bracket_mount:1
- Mate:299: CH_01_0010_syringe_pump_servo:1 ↔ CH_01_0052_bracket_mount:2
- Mate:300: CH_01_0010_syringe_pump_servo:1 ↔ CH_01_0052_bracket_mount:2
- Mate:301: CH_01_0010_syringe_pump_servo:1 ↔ CH_01_0052_bracket_mount:1
- Mate:302: CH_01_0010_syringe_pump_servo:1 ↔ CH_01_0052_bracket_mount:2
- Mate:303: CH_01_0019_bearing_plate_2:1 ↔ CH_01_0053_camera_mount:1
- Flush:53: CH_01_0019_bearing_plate_2:1 ↔ CH_01_0053_camera_mount:1
- Flush:54: CH_01_0019_bearing_plate_2:1 ↔ CH_01_0053_camera_mount:1
- Mate:304: CH_01_0043_camera_PH:1 ↔ CH_01_0054_camer_mount_part_b:1
- Mate:305: CH_01_0043_camera_PH:1 ↔ CH_01_0054_camer_mount_part_b:1
- Mate:306: CH_01_0043_camera_PH:1 ↔ CH_01_0054_camer_mount_part_b:1
- Mate:307: CH_01_0053_camera_mount:1 ↔ CH_01_0054_camer_mount_part_b:1
- Mate:308: CH_01_0053_camera_mount:1 ↔ CH_01_0054_camer_mount_part_b:1
